# Autodesk Inventor assembly: Magnet PanelFrame 90deg connected
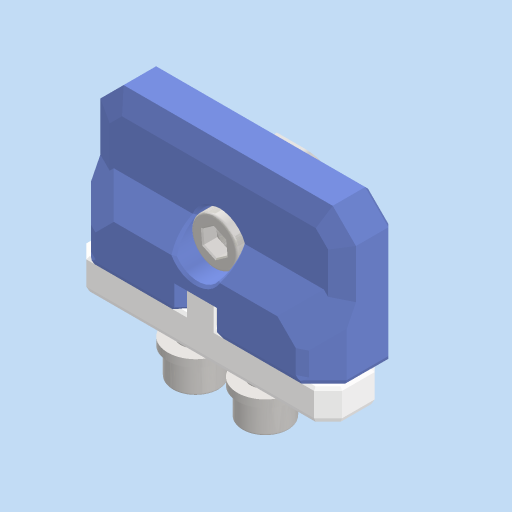
[picture p0: Inventor's stored thumbnail of the model, 512x512]
Saved by Autodesk Inventor 2023.2 (Build 272271000, 271)
## iProperties
Created: 2023-11-30
Part Number: Magnet PanelFrame 90deg connected
Document SubType Name: Assembly
Designer: Nils Bade
Author: Nils Bade
## Documents named in this file (3)
- C:\Users\nilsb\Documents\Inventor\Projektarbeit-Bade\Enclosure\Magnet PanelFrame 90deg connected.iam
- C:\Users\nilsb\Documents\Inventor\Projektarbeit-Bade\Enclosure\Magnet Frame for 4040 - Assembly.iam
- C:\Users\nilsb\Documents\Inventor\Projektarbeit-Bade\Enclosure\Magnet Panel for 4040 - Assembly.iam
## Components (2 placed, 2 different names)
1. Magnet Frame 90deg for 4040 - Assembly:1 [sub-assembly] — Passend:1, Passend:2, Passend:3
2. Magnet Panel for 4040 - Assembly:1 [sub-assembly] — Passend:1, Passend:2, Passend:3
## Relationships (4: Mate 4)
- Passend:1 [Mate]: Magnet Frame 90deg for 4040 - Assembly:1 ↔ Magnet Panel for 4040 - Assembly:1
- Passend:2 [Mate]: Magnet Frame 90deg for 4040 - Assembly:1 ↔ Magnet Panel for 4040 - Assembly:1
- Passend:3 [Mate]: Magnet Frame 90deg for 4040 - Assembly:1 ↔ Magnet Panel for 4040 - Assembly:1
- Passend:5 [Mate]
